# Autodesk Inventor assembly: SmartCube
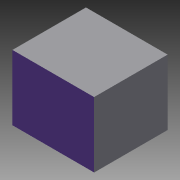
[picture p0: Inventor's stored thumbnail of the model, 180x180]
Saved by Autodesk Inventor 2018.2 (Build 222227000, 227)
## iProperties
Created: 2019-02-06
Part Number: SmartCube
Material: Generisch
Document SubType Name: Assembly
Designer: Lolob
Author: Lolob
## Documents named in this file (9)
- C:\Users\Lolob\Documents\Dipl\Smartcube_Construction\Inventor\SmartCube.iam
- C:\Users\Lolob\Documents\Dipl\Smartcube_Construction\Inventor\Boden.ipt
- C:\Users\Lolob\Documents\Dipl\Smartcube_Construction\Inventor\Wand1.ipt
- C:\Users\Lolob\Documents\Dipl\Smartcube_Construction\Inventor\Wand1_MIR.ipt
- C:\Users\Lolob\Documents\Dipl\Smartcube_Construction\Inventor\Wand2.ipt
- C:\Users\Lolob\Documents\Dipl\Smartcube_Construction\Inventor\Wand2_MIR.ipt
- C:\Users\Lolob\Documents\Dipl\Smartcube_Construction\Inventor\SitzFläche.ipt
- C:\Users\Lolob\Documents\Dipl\Smartcube_Construction\Inventor\Baterie.ipt
- D:\Dokumente\Inventor\Projektname\SitzflächeGlas.ipt
## Components (8 placed, 8 different names)
1. Boden:1 — Passend:1, Passend:2, Passend:3, Starr:1, Starr:2, Starr:4, Passend:7
2. Wand1:1 — Passend:1, Starr:1, Starr:5, Drehbar:1
3. Wand1_MIR:1 — Passend:2, Starr:4
4. Wand2:1 — Drehbar:1
5. Wand2_MIR:1 — Passend:3, Starr:2
6. SitzFläche:1 — Starr:5, Fluchtend:1
7. SitzflächeGlas:1 — Fluchtend:1
8. Baterie:1 — Passend:7
## Relationships (10: Mate 4, WeldJoint 4, RevoluteJoint 1, Flush 1)
- Passend:1 [Mate]: Boden:1 ↔ Wand1:1
- Passend:2 [Mate]: Boden:1 ↔ Wand1_MIR:1
- Passend:3 [Mate]: Boden:1 ↔ Wand2_MIR:1
- Starr:1 [WeldJoint]: Boden:1 ↔ Wand1:1
- Starr:2 [WeldJoint]: Boden:1 ↔ Wand2_MIR:1
- Starr:4 [WeldJoint]: Boden:1 ↔ Wand1_MIR:1
- Starr:5 [WeldJoint]: Wand1:1 ↔ SitzFläche:1
- Drehbar:1 [RevoluteJoint]: Wand1:1 ↔ Wand2:1
- Passend:7 [Mate]: Boden:1 ↔ Baterie:1
- Fluchtend:1 [Flush]: SitzFläche:1 ↔ SitzflächeGlas:1
